# Autodesk Inventor assembly: HingeMK3
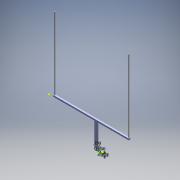
[picture p0: Inventor's stored thumbnail of the model, 180x180]
Saved by Autodesk Inventor 2016 (Build 200138000, 138)
## iProperties
Created: 2017-02-18
Part Number: HingeMK3
Document SubType Name: Assembly
Designer: RoboticsUser
Author: RoboticsUser
## Documents named in this file (5)
- C:\Robotics\CAD\2016-17_CAD\HingeMK3.iam
- C:\Robotics\CAD\2016-17_CAD\HingeMK3Part2.ipt
- C:\Robotics\CAD\2016-17_CAD\slide pivot plate.0001.ipt
- C:\Robotics\CAD\2016-17_CAD\HingeMK3Part3.ipt
- C:\Robotics\CAD\2016-17_CAD\Lift12inBar.ipt
## Components (5 placed, 4 different names)
1. HingeMK3Part2:1 — Mate:1, Mate:3, Mate:4, Flush:1, Mate:5, Tangent:1, Tangent:2, Mate:6, Tangent:3, Tangent:4
2. slide pivot plate.0001:1 — Mate:1, Mate:2, Flush:1
3. HingeMK3Part3:1 — Mate:2, Mate:3, Mate:4
4. Lift12inBar:1 — Mate:6, Tangent:3, Tangent:4
5. Lift12inBar:2 — Mate:5, Tangent:1, Tangent:2
## Relationships (11: Mate 6, Tangent 4, Flush 1)
- Mate:1 (0.5131 mm): HingeMK3Part2:1 ↔ slide pivot plate.0001:1
- Mate:2: slide pivot plate.0001:1 ↔ HingeMK3Part3:1
- Mate:3: HingeMK3Part2:1 ↔ HingeMK3Part3:1
- Mate:4: HingeMK3Part2:1 ↔ HingeMK3Part3:1
- Flush:1: HingeMK3Part2:1 ↔ slide pivot plate.0001:1
- Mate:5: HingeMK3Part2:1 ↔ Lift12inBar:2
- Tangent:1 (1.6002 mm): HingeMK3Part2:1 ↔ Lift12inBar:2
- Tangent:2 (1.6002 mm): HingeMK3Part2:1 ↔ Lift12inBar:2
- Mate:6: HingeMK3Part2:1 ↔ Lift12inBar:1
- Tangent:3 (1.6002 mm): HingeMK3Part2:1 ↔ Lift12inBar:1
- Tangent:4 (1.6002 mm): HingeMK3Part2:1 ↔ Lift12inBar:1
